# Autodesk Inventor assembly: Nozzle
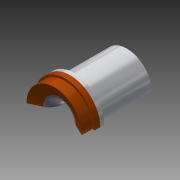
[picture p0: Inventor's stored thumbnail of the model, 180x180]
Saved by Autodesk Inventor 2015 (Build 190159000, 159)
## iProperties
Created: 2016-01-09
Part Number: Nozzle
Document SubType Name: Assembly
Designer: Jared
Author: Jared
## Documents named in this file (4)
- D:\Google Drive\TRC Members\3. IPT (Integrated Product Teams)\Propulsion\2015-2016 Year\6 in Motor\CAD\Flight Motor\Version 3\Nozzle Cut Away.iam
- D:\Google Drive\TRC Members\3. IPT (Integrated Product Teams)\Propulsion\2015-2016 Year\6 in Motor\CAD\Flight Motor\Version 3\Nozzle\Aluminum Carrier.ipt
- D:\Google Drive\TRC Members\3. IPT (Integrated Product Teams)\Propulsion\2015-2016 Year\6 in Motor\CAD\Flight Motor\Version 3\Nozzle\Graphite.ipt
- D:\Google Drive\TRC Members\3. IPT (Integrated Product Teams)\Propulsion\2015-2016 Year\6 in Motor\CAD\Flight Motor\Version 3\Nozzle\Phenolic.ipt
## Components (3 placed, 3 different names)
1. Aluminum Carrier:1 — Mate:2, Mate:6
2. Graphite:1 — Mate:1, Mate:5
3. Phenolic:1 — Mate:1, Mate:2, Mate:5, Mate:6
## Relationships (4: Mate 4)
- Mate:1: Graphite:1 ↔ Phenolic:1
- Mate:2: Aluminum Carrier:1 ↔ Phenolic:1
- Mate:5: Graphite:1 ↔ Phenolic:1
- Mate:6: Aluminum Carrier:1 ↔ Phenolic:1
